# Autodesk Inventor assembly: 2 od flex with versa_MIR
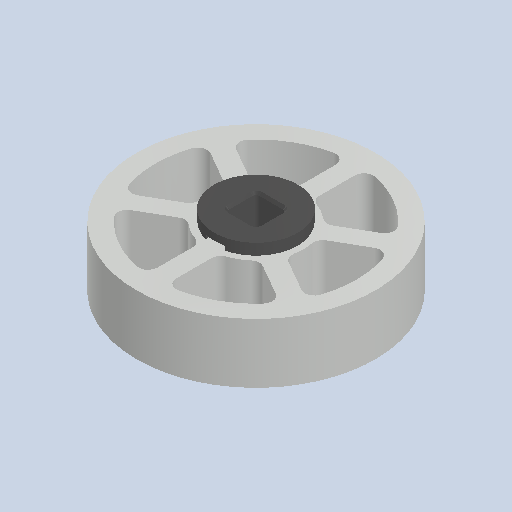
[picture p0: Inventor's stored thumbnail of the model, 512x512]
Saved by Autodesk Inventor 2023 (Build 270158000, 158)
## iProperties
Created: 2022-10-30
Part Number: 2 od flex with versa_MIR
Document SubType Name: Assembly
Designer: aaron
Author: aaron
## Documents named in this file (3)
- C:\Users\aaron\Documents\Inventor\Spin Up\library\Motion\Flex Wheels\2 od flex with versa_MIR.iam
- C:\Users\aaron\Documents\Inventor\Spin Up\library\Motion\Flex Wheels\2.0 OD flex_MIR.ipt
- C:\Users\aaron\Documents\Inventor\Spin Up\library\Motion\Flex Wheels\small versa_MIR.ipt
## Components (3 placed, 2 different names)
1. 2.0 OD flex_MIR:1 — Mate:3, Mate:2, Mate:1
2. small versa_MIR:1 — Mate:3, Flush:2, Flush:1
3. small versa_MIR:2 — Mate:2, Mate:1, Flush:2, Flush:1
## Relationships (5: Mate 3, Flush 2)
- Mate:3: 2.0 OD flex_MIR:1 ↔ small versa_MIR:1
- Mate:2: 2.0 OD flex_MIR:1 ↔ small versa_MIR:2
- Mate:1: 2.0 OD flex_MIR:1 ↔ small versa_MIR:2
- Flush:2: small versa_MIR:1 ↔ small versa_MIR:2
- Flush:1: small versa_MIR:1 ↔ small versa_MIR:2
